# Autodesk Inventor assembly: MotorCapCombinerAssem
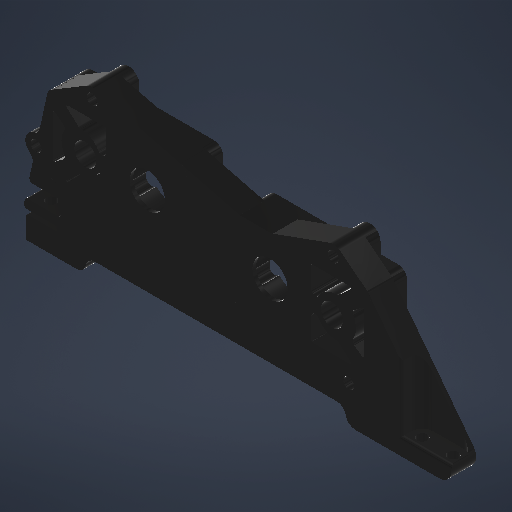
[picture p0: Inventor's stored thumbnail of the model, 512x512]
Saved by Autodesk Inventor 2026.1 (Build 301233000, 233)
## iProperties
Created: 2025-09-08
Part Number: MotorCapCombinerAssem
Document SubType Name: Assembly
Designer: Teddy
Author: Teddy
## Documents named in this file (3)
- C:\Users\Teddy\Desktop\VexCAD\15InVEX\MotorCapCombinerAssem.iam
- C:\Users\Teddy\Desktop\VexCAD\15InVEX\HighMotorMount.ipt
- C:\Users\Teddy\Desktop\VexCAD\15InVEX\CapOGStyle.ipt
## Components (3 placed, 2 different names)
1. HighMotorMount:1 — Flush:1, Flush:2, Mate:1, Mate:2, Mate:3, Mate:4
2. CapOGStyle:1 — Flush:1, Mate:1, Mate:2
3. CapOGStyle:2 — Flush:2, Mate:3, Mate:4
## Relationships (6: Mate 4, Flush 2)
- Flush:1: HighMotorMount:1 ↔ CapOGStyle:1
- Flush:2: HighMotorMount:1 ↔ CapOGStyle:2
- Mate:1 (-0.381 mm): HighMotorMount:1 ↔ CapOGStyle:1
- Mate:2 (-0.381 mm): HighMotorMount:1 ↔ CapOGStyle:1
- Mate:3 (-0.381 mm): HighMotorMount:1 ↔ CapOGStyle:2
- Mate:4 (-0.381 mm): HighMotorMount:1 ↔ CapOGStyle:2
